# Autodesk Inventor assembly: WHE-012 RODAMIENTO
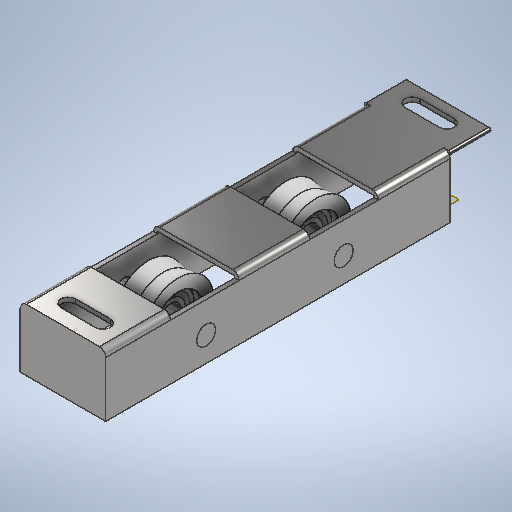
[picture p0: Inventor's stored thumbnail of the model, 512x512]
Saved by Autodesk Inventor 2025 (Build 290162000, 162)
## iProperties
Created: 2026-02-25
Part Number: WHE-012 RODAMIENTO
Document SubType Name: Assembly
Designer: Frank
Author: Frank
## Documents named in this file (5)
- C:\Users\Frank\OneDrive\CARPINTERIA ALUMINIO\PUERTAS Y VENTANAS\ACCESORIOS\RODAMIENTO\WHE-012 RODAMIENTO.iam
- C:\Users\Frank\OneDrive\CARPINTERIA ALUMINIO\PUERTAS Y VENTANAS\ACCESORIOS\RODAMIENTO\CASQUILLO DE RODAMIENTO.ipt
- C:\Users\Frank\OneDrive\CARPINTERIA ALUMINIO\PUERTAS Y VENTANAS\ACCESORIOS\RODAMIENTO\RUEDA.ipt
- C:\Users\Frank\Documents\Inventor\Content Center Files\R2025\es-ES\BS 3469(2)\BS 3469 - 19 - 6 x 15 x 5.ipt
- C:\Users\Frank\OneDrive\CARPINTERIA ALUMINIO\PUERTAS Y VENTANAS\ACCESORIOS\RODAMIENTO\EJE DE RUEDA.ipt
## Components (7 placed, 4 different names)
1. CASQUILLO DE RODAMIENTO:1 — Nivelación:5, Coincidencia:13, Coincidencia:14, Nivelación:6, Coincidencia:15, Coincidencia:16, Nivelación:7, Nivelación:8
2. RUEDA:1 — Coincidencia:1, Nivelación:3, Coincidencia:12, Coincidencia:14
3. BS 3469 (Métrico) 19 - 6 x 15 x 5:1 — Coincidencia:1, Nivelación:3, Coincidencia:2
4. EJE DE RUEDA:1 — Coincidencia:2, Nivelación:5, Coincidencia:13
5. EJE DE RUEDA:2 — Coincidencia:7, Nivelación:6, Coincidencia:15
6. RUEDA:2 — Coincidencia:6, Nivelación:4, Coincidencia:11, Coincidencia:16
7. BS 3469 (Métrico) 19 - 6 x 15 x 5:2 — Coincidencia:6, Nivelación:4, Coincidencia:7
## Relationships (16: Mate 10, Flush 6)
- Coincidencia:1 [Mate]: RUEDA:1 ↔ BS 3469 (Métrico) 19 - 6 x 15 x 5:1
- Nivelación:3 [Flush] (2.25 mm): RUEDA:1 ↔ BS 3469 (Métrico) 19 - 6 x 15 x 5:1
- Coincidencia:2 [Mate]: BS 3469 (Métrico) 19 - 6 x 15 x 5:1 ↔ EJE DE RUEDA:1
- Coincidencia:6 [Mate]: RUEDA:2 ↔ BS 3469 (Métrico) 19 - 6 x 15 x 5:2
- Nivelación:4 [Flush] (2.25 mm): RUEDA:2 ↔ BS 3469 (Métrico) 19 - 6 x 15 x 5:2
- Coincidencia:7 [Mate]: EJE DE RUEDA:2 ↔ BS 3469 (Métrico) 19 - 6 x 15 x 5:2
- Coincidencia:11 [Mate]: RUEDA:2
- Coincidencia:12 [Mate]: RUEDA:1
- Nivelación:5 [Flush]: CASQUILLO DE RODAMIENTO:1 ↔ EJE DE RUEDA:1
- Coincidencia:13 [Mate]: CASQUILLO DE RODAMIENTO:1 ↔ EJE DE RUEDA:1
- Coincidencia:14 [Mate] (7.45 mm): CASQUILLO DE RODAMIENTO:1 ↔ RUEDA:1
- Nivelación:6 [Flush]: CASQUILLO DE RODAMIENTO:1 ↔ EJE DE RUEDA:2
- Coincidencia:15 [Mate]: CASQUILLO DE RODAMIENTO:1 ↔ EJE DE RUEDA:2
- Coincidencia:16 [Mate] (7.45 mm): CASQUILLO DE RODAMIENTO:1 ↔ RUEDA:2
- Nivelación:7 [Flush]: CASQUILLO DE RODAMIENTO:1
- Nivelación:8 [Flush]: CASQUILLO DE RODAMIENTO:1
